# Autodesk Inventor assembly: assembled
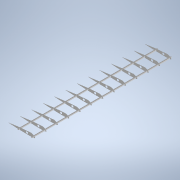
[picture p0: Inventor's stored thumbnail of the model, 180x180]
Saved by Autodesk Inventor 2021 (Build 250183000, 183)
## iProperties
Created: 2021-03-06
Part Number: assembled
Document SubType Name: Assembly
Designer: Ferdinand Hubbard
Author: Ferdinand Hubbard
## Documents named in this file (3)
- C:\Users\Ferdinand Hubbard\Desktop\solarplane\cad\assembled.iam
- C:\Users\Ferdinand Hubbard\Desktop\solarplane\cad\airfoil.ipt
- C:\Users\Ferdinand Hubbard\Desktop\solarplane\cad\centre wood spar.ipt
## Components (15 placed, 2 different names)
1. centre wood spar:1 — Mate:2, Mate:4, Mate:7, Mate:10, Mate:13, Mate:16, Mate:18, Mate:21, Mate:24, Mate:27, Mate:30, Mate:33, Mate:36, Mate:39
2. centre wood spar:2 — Mate:1, Mate:3, Mate:6, Mate:9, Mate:12, Mate:15, Mate:17, Mate:20, Mate:23, Mate:26, Mate:29, Mate:32, Mate:35, Mate:38
3. airfoil:1 — Mate:1, Mate:2, Mate:3, Mate:4, Mate:5
4. airfoil:2 — Mate:5, Mate:6, Mate:7, Mate:8
5. airfoil:3 — Mate:8, Mate:9, Mate:10, Mate:11
6. airfoil:4 — Mate:11, Mate:12, Mate:13, Mate:14
7. airfoil:5 — Mate:14, Mate:15, Mate:16, Mate:19
8. airfoil:6 — Mate:17, Mate:18, Mate:19, Mate:22
9. airfoil:7 — Mate:20, Mate:21, Mate:22, Mate:25
10. airfoil:8 — Mate:23, Mate:24, Mate:25, Mate:28
11. airfoil:9 — Mate:26, Mate:27, Mate:28, Mate:31
12. airfoil:10 — Mate:29, Mate:30, Mate:31, Mate:34
13. airfoil:11 — Mate:32, Mate:33, Mate:34, Mate:37
14. airfoil:12 — Mate:35, Mate:36, Mate:37, Mate:40
15. airfoil:13 — Mate:38, Mate:39, Mate:40
## Relationships (40: Mate 40)
- Mate:1: centre wood spar:2 ↔ airfoil:1
- Mate:2: centre wood spar:1 ↔ airfoil:1
- Mate:3 (20 mm): centre wood spar:2 ↔ airfoil:1
- Mate:4 (20 mm): centre wood spar:1 ↔ airfoil:1
- Mate:5 (156.5 mm): airfoil:1 ↔ airfoil:2
- Mate:6: centre wood spar:2 ↔ airfoil:2
- Mate:7: centre wood spar:1 ↔ airfoil:2
- Mate:8 (156.5 mm): airfoil:2 ↔ airfoil:3
- Mate:9: centre wood spar:2 ↔ airfoil:3
- Mate:10: centre wood spar:1 ↔ airfoil:3
- Mate:11 (156.5 mm): airfoil:3 ↔ airfoil:4
- Mate:12: centre wood spar:2 ↔ airfoil:4
- Mate:13: centre wood spar:1 ↔ airfoil:4
- Mate:14 (156.5 mm): airfoil:4 ↔ airfoil:5
- Mate:15: centre wood spar:2 ↔ airfoil:5
- Mate:16: centre wood spar:1 ↔ airfoil:5
- Mate:17: centre wood spar:2 ↔ airfoil:6
- Mate:18: centre wood spar:1 ↔ airfoil:6
- Mate:19 (156.5 mm): airfoil:5 ↔ airfoil:6
- Mate:20: centre wood spar:2 ↔ airfoil:7
- Mate:21: centre wood spar:1 ↔ airfoil:7
- Mate:22 (156.5 mm): airfoil:6 ↔ airfoil:7
- Mate:23: centre wood spar:2 ↔ airfoil:8
- Mate:24: centre wood spar:1 ↔ airfoil:8
- Mate:25 (156.5 mm): airfoil:7 ↔ airfoil:8
- Mate:26: centre wood spar:2 ↔ airfoil:9
- Mate:27: centre wood spar:1 ↔ airfoil:9
- Mate:28 (156.5 mm): airfoil:8 ↔ airfoil:9
- Mate:29: centre wood spar:2 ↔ airfoil:10
- Mate:30: centre wood spar:1 ↔ airfoil:10
- Mate:31 (156.5 mm): airfoil:9 ↔ airfoil:10
- Mate:32: centre wood spar:2 ↔ airfoil:11
- Mate:33: centre wood spar:1 ↔ airfoil:11
- Mate:34 (156.5 mm): airfoil:10 ↔ airfoil:11
- Mate:35: centre wood spar:2 ↔ airfoil:12
- Mate:36: centre wood spar:1 ↔ airfoil:12
- Mate:37 (156.5 mm): airfoil:11 ↔ airfoil:12
- Mate:38: centre wood spar:2 ↔ airfoil:13
- Mate:39: centre wood spar:1 ↔ airfoil:13
- Mate:40 (156.5 mm): airfoil:12 ↔ airfoil:13
